# Autodesk Inventor assembly: 3A.01.12.JS.Rib 12
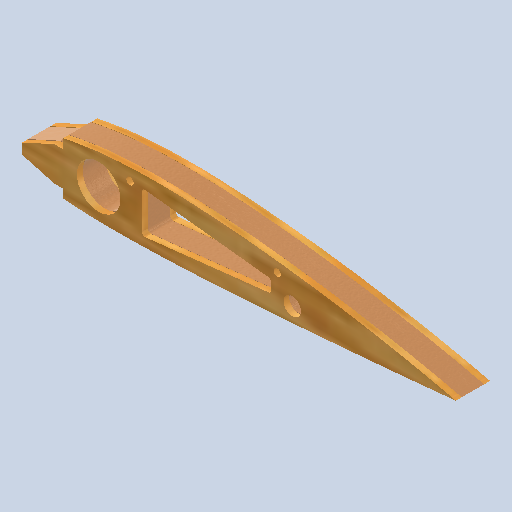
[picture p0: Inventor's stored thumbnail of the model, 512x512]
Saved by Autodesk Inventor 2025.1 (Build 291241000, 241)
## iProperties
Created: 2025-01-14
Part Number: 3A.01.12.JS.Rib 12
Document SubType Name: Assembly
Designer: johan
Author: johan
## Documents named in this file (3)
- C:\Users\johan\OneDrive - University of Bristol\CAD docs\2) Wing\2) Ribs\assemblies\3A.01.12.JS.Rib 12.iam
- C:\Users\johan\OneDrive - University of Bristol\CAD docs\2) Wing\2) Ribs\parts\Full length unmodified\3P.03.12.01.JS.rib 12 ply.ipt
- C:\Users\johan\OneDrive - University of Bristol\CAD docs\2) Wing\2) Ribs\parts\Full length unmodified\3P.03.12.02.JS.rib 12 foam.ipt
## Components (3 placed, 2 different names)
1. 3P.03.12.01.JS.rib 12 ply:1 — Rigid:2
2. 3P.03.12.02.JS.rib 12 foam:1 — Rigid:1, Rigid:2
3. 3P.03.12.01.JS.rib 12 ply:2 — Rigid:1
## Relationships (2: WeldJoint 2)
- Rigid:1 [WeldJoint]: 3P.03.12.02.JS.rib 12 foam:1 ↔ 3P.03.12.01.JS.rib 12 ply:2
- Rigid:2 [WeldJoint]: 3P.03.12.01.JS.rib 12 ply:1 ↔ 3P.03.12.02.JS.rib 12 foam:1
